# Autodesk Inventor assembly: RobotPallet
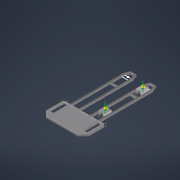
[picture p0: Inventor's stored thumbnail of the model, 180x180]
Saved by Autodesk Inventor 2022 (Build 260153000, 153)
## iProperties
Created: 2021-09-10
Part Number: RobotPallet
Material: Generic
Document SubType Name: Assembly
Designer: Andres
Author: Andres
## Documents named in this file (5)
- D:\Documentos\15.PUCP_2021-2\[PDM] Proyecto de Diseño Mecatrónico\ProyectoGIT\ProyectoRobotPallet\RobotPallet.iam
- D:\Documentos\15.PUCP_2021-2\[PDM] Proyecto de Diseño Mecatrónico\ProyectoGIT\ProyectoRobotPallet\Estructura Inferior\EstructuraInferior.iam
- D:\Documentos\15.PUCP_2021-2\[PDM] Proyecto de Diseño Mecatrónico\ProyectoGIT\ProyectoRobotPallet\Estructura Inferior\PlanchaBaseInferior.ipt
- D:\Documentos\15.PUCP_2021-2\[PDM] Proyecto de Diseño Mecatrónico\ProyectoGIT\ProyectoRobotPallet\SistemaDeElevacion\version2\SistemaElevacionV2.iam
- SistemaElevacion2.iam
## Components (4 placed, 3 different names)
1. EstructuraInferior:1 [sub-assembly] — Flush:1, Mate:1, Flush:2, Mate:2, Flush:3
2. PlanchaBaseInferior:1 — Flush:1
3. SistemaElevacion2:1 [sub-assembly] — Mate:1, Flush:2, Mate:3
4. SistemaElevacion2:2 [sub-assembly] — Mate:2, Flush:3, Mate:3
## Relationships (6: Flush 3, Mate 3)
- Flush:1: EstructuraInferior:1 ↔ PlanchaBaseInferior:1
- Mate:1: EstructuraInferior:1 ↔ SistemaElevacion2:1
- Flush:2: EstructuraInferior:1 ↔ SistemaElevacion2:1
- Mate:2: EstructuraInferior:1 ↔ SistemaElevacion2:2
- Flush:3: EstructuraInferior:1 ↔ SistemaElevacion2:2
- Mate:3 (800 mm): SistemaElevacion2:1 ↔ SistemaElevacion2:2
